# Autodesk Inventor assembly: !tower
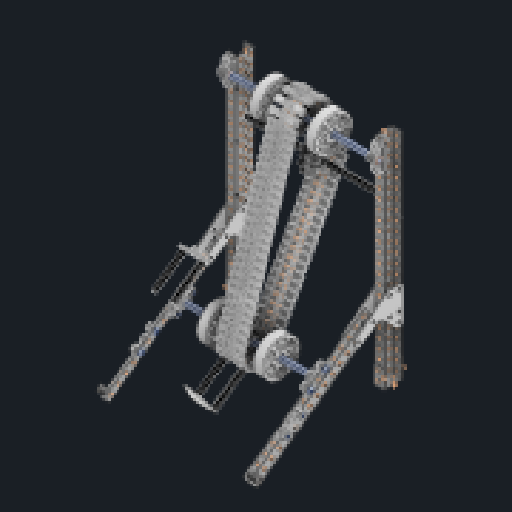
[picture p0: Inventor's stored thumbnail of the model, 512x512]
Saved by Autodesk Inventor 2025 (Build 290162000, 162)
## iProperties
Created: 2024-10-13
Part Number: !tower
Document SubType Name: Assembly
Designer: Averey Ku
Author: Averey Ku
## Documents named in this file (21)
- D:\vex_robotics_high_stakes\hardware\cad\bots\high_stakes_v2\tower\!tower.iam
- D:\vex_robotics_high_stakes\hardware\cad\bots\high_stakes_v2\tower\structure\!structure.iam
- D:\vex_robotics_high_stakes\hardware\cad\robpros_cad_lib\Motion\Shaft HS\Shaft HS\Shaft HS 7.5 in.ipt
- D:\vex_robotics_high_stakes\hardware\cad\robpros_cad_lib\Motion\Shaft HS\Shaft HS.ipt
- D:\vex_robotics_high_stakes\hardware\cad\robpros_cad_lib\Motion\Sprockets\9P Sprocket.iam
- D:\vex_robotics_high_stakes\hardware\cad\robpros_cad_lib\Motion\Sprockets\9P Sprocket\9P 12T Sprocket, No Insert.iam
- D:\vex_robotics_high_stakes\hardware\cad\robpros_cad_lib\Motion\Wheels\Flex Wheels\2.000 Flex Wheel\2.000 30A .500.ipt
- D:\vex_robotics_high_stakes\hardware\cad\robpros_cad_lib\Motion\Wheels\Flex Wheels\2.000 Flex Wheel.ipt
- D:\vex_robotics_high_stakes\hardware\cad\robpros_cad_lib\Motion\Shaft HS\Shaft HS\Shaft HS 8.5 in.ipt
- D:\vex_robotics_high_stakes\hardware\cad\bots\high_stakes_v2\tower\chain_path.ipt
- D:\vex_robotics_high_stakes\hardware\cad\robpros_cad_lib\Motion\Chain 9P\Tank Tread Traction Link.ipt
- D:\vex_robotics_high_stakes\hardware\cad\robpros_cad_lib\Motion\Chain 9P\Chain Attachment Link.ipt
- D:\vex_robotics_high_stakes\hardware\cad\robpros_cad_lib\Structure\Standoff\Standoff .25.ipt
- D:\vex_robotics_high_stakes\hardware\cad\robpros_cad_lib\Structure\Standoff.ipt
- D:\vex_robotics_high_stakes\hardware\cad\robpros_cad_lib\Structure\Standoff\Standoff 3.00.ipt
- D:\vex_robotics_high_stakes\hardware\cad\robpros_cad_lib\Motion\Spacers\Spacer Nylon .375 OD\NSpacer .375 OD x .125.ipt
- D:\vex_robotics_high_stakes\hardware\cad\robpros_cad_lib\Motion\Spacers\Spacer Nylon .375 OD.ipt
- D:\vex_robotics_high_stakes\hardware\cad\robpros_cad_lib\Motion\Spacers\Washer Steel\SWasher .375 OD x .031250.ipt
- D:\vex_robotics_high_stakes\hardware\cad\robpros_cad_lib\Motion\Spacers\Washer Steel.ipt
- D:\vex_robotics_high_stakes\hardware\cad\robpros_cad_lib\Structure\Standoff\Standoff 2.00.ipt
- D:\vex_robotics_high_stakes\hardware\cad\bots\high_stakes_v2\intake\custom_parts\hook_gusset.ipt
## Components (95 placed, 14 different names)
1. !structure:1 [sub-assembly] — Insert:1, Insert:2, Insert:5, Insert:11, Insert:17
2. Shaft HS 7.5 in:1 — Insert:1
3. 9P 12T Sprocket, No Insert:2 [sub-assembly] — Insert:2, Insert:3, Insert:4, Flush:1, Flush:3
4. 2.000 30A .500:1 — Insert:3
5. 2.000 30A .500:2 — Insert:4
6. Shaft HS 8.5 in:2 — Insert:5, Mate:1
7. 9P 12T Sprocket, No Insert:3 [sub-assembly] — Flush:1, Mate:1, Insert:6, Insert:7, Flush:2, Mate:3
8. 2.000 30A .500:3 — Insert:6
9. 2.000 30A .500:4 — Insert:7
10. 9P 12T Sprocket, No Insert:4 [sub-assembly] — Flush:2
11. chain_path:1 — Flush:3, Mate:4, Angle:1
12. Chain Attachment Link:1 — Insert:9, Mate:5
13. Standoff .25:1 — Insert:10, Insert:13
14. Standoff 3.00:2 — Insert:10, Insert:11
15. NSpacer .375 OD x .125:1 — Insert:12, Insert:13
16. SWasher .375 OD x .031250:1 — Insert:12
17. Standoff .25:3
18. Standoff 3.00:4 — Insert:17
19. NSpacer .375 OD x .125:2
20. SWasher .375 OD x .031250:2
21. Standoff 2.00:7 — Mate:9
22. Standoff 2.00:8 — Insert:25
23. Chain Attachment Link:3 — Insert:24, Mate:8
24. hook_gusset:2 — Insert:25, Mate:9
25. Standoff 2.00:9
26. Standoff 2.00:10
27. Chain Attachment Link:4 — Insert:29, Mate:11
28. hook_gusset:3
29. Standoff 2.00:11
30. Standoff 2.00:12
31. Chain Attachment Link:5 — Insert:33, Mate:13
32. hook_gusset:4
33. Tank Tread Traction Link:1 — Mate:3, Mate:4, Angle:1
34. Tank Tread Traction Link:2
35. Tank Tread Traction Link:3
36. Tank Tread Traction Link:4
37. Tank Tread Traction Link:5
38. Tank Tread Traction Link:6
39. Tank Tread Traction Link:7
40. Tank Tread Traction Link:8
41. Tank Tread Traction Link:9
42. Tank Tread Traction Link:10
43. Tank Tread Traction Link:11
44. Tank Tread Traction Link:12
45. Tank Tread Traction Link:13
46. Tank Tread Traction Link:14
47. Tank Tread Traction Link:15
48. Tank Tread Traction Link:16
49. Tank Tread Traction Link:17
50. Tank Tread Traction Link:18
51. Tank Tread Traction Link:19 — Insert:33, Mate:13
52. Tank Tread Traction Link:20
53. Tank Tread Traction Link:21
54. Tank Tread Traction Link:22
55. Tank Tread Traction Link:23
56. Tank Tread Traction Link:24
57. Tank Tread Traction Link:25
58. Tank Tread Traction Link:26
59. Tank Tread Traction Link:27
60. Tank Tread Traction Link:28
61. Tank Tread Traction Link:29
62. Tank Tread Traction Link:30
63. Tank Tread Traction Link:31
64. Tank Tread Traction Link:32
65. Tank Tread Traction Link:33
66. Tank Tread Traction Link:34
67. Tank Tread Traction Link:35
68. Tank Tread Traction Link:36
69. Tank Tread Traction Link:37
70. Tank Tread Traction Link:38
71. Tank Tread Traction Link:39
72. Tank Tread Traction Link:40 — Insert:29, Mate:11
73. Tank Tread Traction Link:41
74. Tank Tread Traction Link:42
75. Tank Tread Traction Link:43
76. Tank Tread Traction Link:44
77. Tank Tread Traction Link:45
78. Tank Tread Traction Link:46
79. Tank Tread Traction Link:47
80. Tank Tread Traction Link:48
81. Tank Tread Traction Link:49
82. Tank Tread Traction Link:50
83. Tank Tread Traction Link:51
84. Tank Tread Traction Link:52
85. Tank Tread Traction Link:53 — Insert:9, Mate:5
86. Tank Tread Traction Link:54
87. Tank Tread Traction Link:55
88. Tank Tread Traction Link:56
89. Tank Tread Traction Link:57
90. Tank Tread Traction Link:58
91. Tank Tread Traction Link:59
92. Tank Tread Traction Link:60
93. Tank Tread Traction Link:61 — Insert:24, Mate:8
94. Tank Tread Traction Link:62
95. Tank Tread Traction Link:63
## Component patterns: (63 elements, first: Tank Tread Traction Link:1)
## Relationships (42: Insert 28, Mate 10, Flush 3, Angle 1)
- Insert:1: !structure:1 ↔ Shaft HS 7.5 in:1
- Insert:2 (87.9094 mm): !structure:1 ↔ 9P 12T Sprocket, No Insert:2
- Insert:3 (25.4 mm): 9P 12T Sprocket, No Insert:2 ↔ 2.000 30A .500:1
- Insert:4 (25.4 mm): 9P 12T Sprocket, No Insert:2 ↔ 2.000 30A .500:2
- Insert:5: !structure:1 ↔ Shaft HS 8.5 in:2
- Flush:1: 9P 12T Sprocket, No Insert:2 ↔ 9P 12T Sprocket, No Insert:3
- Mate:1: Shaft HS 8.5 in:2 ↔ 9P 12T Sprocket, No Insert:3
- Insert:6 (25.4 mm): 9P 12T Sprocket, No Insert:3 ↔ 2.000 30A .500:3
- Insert:7 (25.4 mm): 9P 12T Sprocket, No Insert:3 ↔ 2.000 30A .500:4
- Flush:2: 9P 12T Sprocket, No Insert:3 ↔ 9P 12T Sprocket, No Insert:4
- Flush:3: 9P 12T Sprocket, No Insert:2 ↔ chain_path:1
- Mate:3: 9P 12T Sprocket, No Insert:3 ↔ Tank Tread Traction Link:1
- Mate:4: chain_path:1 ↔ Tank Tread Traction Link:1
- Angle:1 (-90 deg): chain_path:1 ↔ Tank Tread Traction Link:1
- Insert:9: Chain Attachment Link:1 ↔ Tank Tread Traction Link:53
- Mate:5: Chain Attachment Link:1 ↔ Tank Tread Traction Link:53
- Insert:10: Standoff .25:1 ↔ Standoff 3.00:2
- Insert:11: !structure:1 ↔ Standoff 3.00:2
- Insert:12: NSpacer .375 OD x .125:1 ↔ SWasher .375 OD x .031250:1
- Insert:13: Standoff .25:1 ↔ NSpacer .375 OD x .125:1
- [Insert]: Standoff .25:3 ↔ Standoff 3.00:4
- [Insert]: NSpacer .375 OD x .125:2 ↔ SWasher .375 OD x .031250:2
- [Insert]: Standoff .25:3 ↔ NSpacer .375 OD x .125:2
- Insert:17: !structure:1 ↔ Standoff 3.00:4
- [Insert]: Standoff 2.00:8 ↔ Chain Attachment Link:3
- [Insert]: Standoff 2.00:7 ↔ Chain Attachment Link:3
- Insert:24: Chain Attachment Link:3 ↔ Tank Tread Traction Link:61
- Mate:8: Chain Attachment Link:3 ↔ Tank Tread Traction Link:61
- Insert:25: Standoff 2.00:8 ↔ hook_gusset:2
- Mate:9: Standoff 2.00:7 ↔ hook_gusset:2
- [Insert]: Standoff 2.00:10 ↔ Chain Attachment Link:4
- [Insert]: Standoff 2.00:9 ↔ Chain Attachment Link:4
- [Insert]: Standoff 2.00:10 ↔ hook_gusset:3
- [Mate]: Standoff 2.00:9 ↔ hook_gusset:3
- Insert:29: Chain Attachment Link:4 ↔ Tank Tread Traction Link:40
- Mate:11: Chain Attachment Link:4 ↔ Tank Tread Traction Link:40
- [Insert]: Standoff 2.00:12 ↔ Chain Attachment Link:5
- [Insert]: Standoff 2.00:11 ↔ Chain Attachment Link:5
- [Insert]: Standoff 2.00:12 ↔ hook_gusset:4
- [Mate]: Standoff 2.00:11 ↔ hook_gusset:4
- Insert:33: Chain Attachment Link:5 ↔ Tank Tread Traction Link:19
- Mate:13: Chain Attachment Link:5 ↔ Tank Tread Traction Link:19
## Named parameters: d31_d27 = 0 mm, d32_d29 = 0 mm, d33_d30 = 0 mm, d45_d35 = 0 mm, d46_d36 = 0 mm, d51_d45_d35 = 0 mm, d52_d46_d36 = 0 mm, d53_d49 = 0 mm, d54_d50 = 0 mm, d57_d51_d45_d35 = 0 mm, d58_d52_d46_d36 = 0 mm, d59_d53_d49 = 0 mm, d60_d54_d50 = 0 mm
